# Autodesk Inventor assembly: PayloadGermination
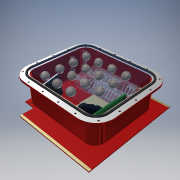
[picture p0: Inventor's stored thumbnail of the model, 180x180]
Saved by Autodesk Inventor 2018 (Build 220112000, 112)
## iProperties
Created: 2018-07-04
Part Number: PayloadGermination
Document SubType Name: Assembly
Designer: Bradley
Mass: 89.3017 g
Surface Area: 529.298 cm^2
Volume: 39.4669 cm^3
Density: 2.2627 g/cm^3
Author: Bradley
## Documents named in this file (18)
- D:\Users\Bradley\Documents\CougsInSpace\CougSat1-Hardware\CougSat1-Payload\CADModel\Native\PayloadGermination.iam
- D:\Users\Bradley\Documents\CougsInSpace\CougSat1-Hardware\CougSat1-Payload\CADModel\Native\PayloadGermination_PCB.ipt
- D:\Users\Bradley\Documents\CougsInSpace\CougSat1-Hardware\CougSat1-Payload\CADModel\Native\PayloadGermination_Chamber.ipt
- D:\Users\Bradley\Documents\CougsInSpace\Resources\ComponentModels\Electronics\Module_ArducamMini.ipt
- D:\Users\Bradley\Documents\CougsInSpace\CougSat1-Hardware\CougSat1-Payload\CADModel\Native\PayloadGermination_Mirror.ipt
- D:\Users\Bradley\Documents\CougsInSpace\CougSat1-Hardware\CougSat1-Payload\CADModel\Native\PayloadGermination_Seal.ipt
- D:\Users\Bradley\Documents\CougsInSpace\Resources\ComponentModels\Hardware\Lens_M12_1.70mm-f2.8.ipt
- D:\Users\Bradley\Documents\CougsInSpace\Resources\ComponentModels\Hardware\LensMount_M12-20mm.ipt
- D:\Users\Bradley\Documents\CougsInSpace\Resources\ComponentModels\Electronics\Module_CO2Sensor-T6713.ipt
- D:\Users\Bradley\Documents\CougsInSpace\CougSat1-Hardware\CougSat1-Payload\CADModel\Native\PayloadGermination_Seed.ipt
- D:\Users\Bradley\Documents\CougsInSpace\CougSat1-Hardware\CougSat1-Payload\CADModel\Native\PayloadGermination_Sponge.ipt
- D:\Users\Bradley\Documents\CougsInSpace\CougSat1-Hardware\CougSat1-Payload\CADModel\Native\PayloadGermination_Syringe.ipt
- D:\Users\Bradley\Documents\CougsInSpace\Resources\ComponentModels\Hardware\Spring_11x39mm.ipt
- D:\Users\Bradley\Documents\CougsInSpace\CougSat1-Hardware\CougSat1-Payload\CADModel\Native\PayloadGermination_SyringeCap.ipt
- D:\Users\Bradley\Documents\CougsInSpace\CougSat1-Hardware\CougSat1-Payload\CADModel\Native\PayloadGermination_SyringePlunger.ipt
- D:\Users\Bradley\Documents\CougsInSpace\Resources\ComponentModels\Hardware\ORing_1x10mm.ipt
- D:\Users\Bradley\Documents\CougsInSpace\Resources\ComponentModels\Electronics\Resistor_TH-15mm.ipt
- D:\Users\Bradley\Documents\CougsInSpace\CougSat1-Hardware\CougSat1-Payload\CADModel\Native\PayloadGermination_SyringeTube.ipt
## Components (38 placed, 17 different names)
1. PayloadGermination_PCB:1
2. PayloadGermination_Chamber:1 — Flush:1, Flush:2, Flush:3, Mate:1, Mate:2, Insert:1, Insert:2, Mate:3, Insert:6, Insert:7, Flush:6, Flush:10, Angle:1
3. Module_ArducamMini:1 — Mate:1, Mate:2, Insert:3, Insert:4, Insert:5, Mate:4
4. PayloadGermination_Mirror:1
5. PayloadGermination_Seal:1 — Insert:1, Insert:2
6. Lens_M12_1.70mm-f2.8:1 — Insert:5
7. LensMount_M12-20mm:1 — Insert:3, Insert:4
8. Module_CO2Sensor-T6713:1 — Mate:3, Mate:4
9. PayloadGermination_Seed:2
10. PayloadGermination_Seed:3
11. PayloadGermination_Seed:4
12. PayloadGermination_Seed:6
13. PayloadGermination_Seed:7
14. PayloadGermination_Seed:8
15. PayloadGermination_Seed:9
16. PayloadGermination_Seed:10
17. PayloadGermination_Seed:11
18. PayloadGermination_Seed:12
19. PayloadGermination_Seed:13
20. PayloadGermination_Seed:14
21. PayloadGermination_Seed:15
22. PayloadGermination_Seed:5
23. PayloadGermination_Seed:1
24. PayloadGermination_Sponge:1 — Insert:6, Insert:7
25. PayloadGermination_Syringe:1 — Insert:8, Mate:5, Insert:9, Flush:6, Flush:7, Flush:8, Insert:12
26. Spring_11x39mm:1 — Flush:4, Mate:5
27. PayloadGermination_SyringeCap:1 — Insert:8, Flush:4, Mate:8, Mate:9
28. PayloadGermination_SyringePlunger:1 — Mate:6, Mate:7, Insert:9
29. ORing_1x10mm:1 — Mate:6, Mate:7
30. Resistor_TH-15mm:1 — Mate:8, Mate:9
31. PayloadGermination_Syringe:2 — Flush:9, Flush:10, Mate:15, Insert:13
32. Spring_11x39mm:2
33. PayloadGermination_SyringeCap:2
34. PayloadGermination_SyringePlunger:2
35. ORing_1x10mm:2
36. Resistor_TH-15mm:2
37. PayloadGermination_SyringeTube:1 — Insert:13, Angle:1, Angle:2
38. PayloadGermination_SyringeTube:2 — Insert:12, Angle:2
## Relationships (40: Mate 15, Insert 13, Flush 10, Angle 2)
- Flush:1: PayloadGermination_Chamber:1
- Flush:2 (-31.5 mm): PayloadGermination_Chamber:1
- Flush:3 (44.4 mm): PayloadGermination_Chamber:1
- Mate:1: PayloadGermination_Chamber:1 ↔ Module_ArducamMini:1
- Mate:2 (5 mm): PayloadGermination_Chamber:1 ↔ Module_ArducamMini:1
- Insert:1: PayloadGermination_Chamber:1 ↔ PayloadGermination_Seal:1
- Insert:2: PayloadGermination_Chamber:1 ↔ PayloadGermination_Seal:1
- Insert:3: Module_ArducamMini:1 ↔ LensMount_M12-20mm:1
- Insert:4: Module_ArducamMini:1 ↔ LensMount_M12-20mm:1
- Insert:5: Module_ArducamMini:1 ↔ Lens_M12_1.70mm-f2.8:1
- Mate:3: PayloadGermination_Chamber:1 ↔ Module_CO2Sensor-T6713:1
- Mate:4 (5 mm): Module_ArducamMini:1 ↔ Module_CO2Sensor-T6713:1
- Insert:6: PayloadGermination_Chamber:1 ↔ PayloadGermination_Sponge:1
- Insert:7: PayloadGermination_Chamber:1 ↔ PayloadGermination_Sponge:1
- Insert:8: PayloadGermination_Syringe:1 ↔ PayloadGermination_SyringeCap:1
- Flush:4 (-0.5 mm): Spring_11x39mm:1 ↔ PayloadGermination_SyringeCap:1
- Mate:5: PayloadGermination_Syringe:1 ↔ Spring_11x39mm:1
- Mate:6: PayloadGermination_SyringePlunger:1 ↔ ORing_1x10mm:1
- Mate:7 (0.5 mm): PayloadGermination_SyringePlunger:1 ↔ ORing_1x10mm:1
- Insert:9: PayloadGermination_Syringe:1 ↔ PayloadGermination_SyringePlunger:1
- Mate:8 (2 mm): PayloadGermination_SyringeCap:1 ↔ Resistor_TH-15mm:1
- Mate:9: PayloadGermination_SyringeCap:1 ↔ Resistor_TH-15mm:1
- [Insert]: PayloadGermination_Syringe:2 ↔ PayloadGermination_SyringeCap:2
- [Flush] (-0.5 mm): Spring_11x39mm:2 ↔ PayloadGermination_SyringeCap:2
- [Mate]: PayloadGermination_Syringe:2 ↔ Spring_11x39mm:2
- [Mate]: PayloadGermination_SyringePlunger:2 ↔ ORing_1x10mm:2
- [Mate] (0.5 mm): PayloadGermination_SyringePlunger:2 ↔ ORing_1x10mm:2
- [Insert]: PayloadGermination_Syringe:2 ↔ PayloadGermination_SyringePlunger:2
- [Mate] (2 mm): PayloadGermination_SyringeCap:2 ↔ Resistor_TH-15mm:2
- [Mate]: PayloadGermination_SyringeCap:2 ↔ Resistor_TH-15mm:2
- Flush:6 (-9 mm): PayloadGermination_Chamber:1 ↔ PayloadGermination_Syringe:1
- Flush:7 (-46 mm): PayloadGermination_Syringe:1
- Flush:8 (-25 mm): PayloadGermination_Syringe:1
- Flush:9 (-46 mm): PayloadGermination_Syringe:2
- Flush:10 (-9 mm): PayloadGermination_Chamber:1 ↔ PayloadGermination_Syringe:2
- Mate:15 (10 mm): PayloadGermination_Syringe:2
- Insert:12: PayloadGermination_Syringe:1 ↔ PayloadGermination_SyringeTube:2
- Insert:13: PayloadGermination_Syringe:2 ↔ PayloadGermination_SyringeTube:1
- Angle:1 (0 deg): PayloadGermination_Chamber:1 ↔ PayloadGermination_SyringeTube:1
- Angle:2 (0 deg): PayloadGermination_SyringeTube:1 ↔ PayloadGermination_SyringeTube:2
## Named parameters: d29_d23 = 0 mm, d30_d24 = 28 mm, d31_d25 = 0 mm, d32_d26 = 2 mm, d33_d27 = 0 mm, d34_d18 = 0 mm, d35_d19 = -0.5 mm, d36_d20 = 0 mm, d37_d21 = 0 mm, d38_d22 = 0.5 mm
